# Autodesk Inventor assembly: Assembly_Cube_28byi_Motor_v3
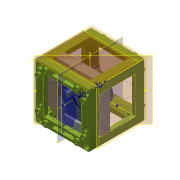
[picture p0: Inventor's stored thumbnail of the model, 180x180]
Saved by Autodesk Inventor 2019.4 (Build 234330000, 330)
## iProperties
Created: 2019-07-23
Part Number: Assembly_Cube_28byi_Motor_v3
Document SubType Name: Assembly
Designer: marsikovabarbora
Mass: 41.4978 g
Surface Area: 307.795 cm^2
Volume: 37.4817 cm^3
Density: 1.10715 g/cm^3
Author: marsikovabarbora
## Documents named in this file (4)
- C:\Users\diederichbenedict\Dropbox\Dokumente\Promotion\PROJECTS\UC2\02_CAD\INVENTOR\uc2_v3\Assembly_Cube_28byi_Motor_v3.iam
- C:\Users\diederichbenedict\Dropbox\Dokumente\Promotion\PROJECTS\UC2\02_CAD\INVENTOR\uc2_v3\Assembly_Cube_empty_IM_v3.iam
- C:\Users\diederichbenedict\Dropbox\Dokumente\Promotion\PROJECTS\UC2\02_CAD\INVENTOR\uc2_v3\00_Stepper_Motor_28BYJ-48.ipt
- C:\Users\diederichbenedict\Dropbox\Dokumente\Promotion\PROJECTS\UC2\02_CAD\INVENTOR\uc2_v3\20_Cube_Insert_StepperMotor_28byi_v3.ipt
## Components (3 placed, 3 different names)
1. Assembly_Cube_empty_IM_v3:1 [sub-assembly] — Mate:1, Mate:2, Mate:5, Mate:10, Mate:11, Angle:1, Flush:1, Flush:2
2. 00_Stepper_Motor_28BYJ-48:1 — Mate:10, Mate:11, Angle:1
3. 20_Cube_Insert_StepperMotor_28byi_v3:1 — Flush:1, Flush:2
## Relationships (8: Mate 5, Flush 2, Angle 1)
- Mate:1: Assembly_Cube_empty_IM_v3:1
- Mate:2: Assembly_Cube_empty_IM_v3:1
- Mate:5: Assembly_Cube_empty_IM_v3:1
- Mate:10 (10 mm): Assembly_Cube_empty_IM_v3:1 ↔ 00_Stepper_Motor_28BYJ-48:1
- Mate:11: Assembly_Cube_empty_IM_v3:1 ↔ 00_Stepper_Motor_28BYJ-48:1
- Angle:1 (0 deg): Assembly_Cube_empty_IM_v3:1 ↔ 00_Stepper_Motor_28BYJ-48:1
- Flush:1: Assembly_Cube_empty_IM_v3:1 ↔ 20_Cube_Insert_StepperMotor_28byi_v3:1
- Flush:2: Assembly_Cube_empty_IM_v3:1 ↔ 20_Cube_Insert_StepperMotor_28byi_v3:1
